# Autodesk Inventor assembly: Top Rail assy
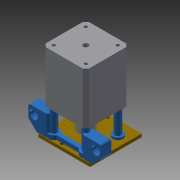
[picture p0: Inventor's stored thumbnail of the model, 180x180]
Saved by Autodesk Inventor 2013 SP2 (Build 170200200, 200)
## iProperties
Created: 2017-01-25
Part Number: Top Rail assy
Document SubType Name: Assembly
Designer: Herman de Vries
Mass: 171.449 g
Surface Area: 753.144 cm^2
Volume: 171.449 cm^3
Density: 1 g/cm^3
Author: Herman de Vries
## Documents named in this file (6)
- C:\Users\hdv\Dropbox\Projects\Inventor\PaintBot_3\Top Rail assy.iam
- C:\Users\hdv\Dropbox\Projects\Inventor\PaintBot_3\Top Rail.ipt
- C:\Users\hdv\Dropbox\Projects\Inventor\PaintBot_3\NEMA42.ipt
- C:\Users\hdv\Dropbox\Projects\Inventor\PaintBot_3\gear belt.ipt
- C:\Users\hdv\Dropbox\Projects\Inventor\PaintBot_3\spacer stepperM.ipt
- C:\Users\hdv\Dropbox\Projects\Inventor\PaintBot_3\spacer stepperM n rail.ipt
## Components (6 placed, 5 different names)
1. Top Rail:1 — Mate:1, Mate:3
2. NEMA42:1 — Insert:1, Mate:1, Mate:3, Insert:5
3. gear belt:1 — Insert:1
4. spacer stepperM:1
5. spacer stepperM:2
6. spacer stepperM n rail:1 — Insert:5
## Relationships (7: Insert 5, Mate 2)
- Insert:1 (5 mm): NEMA42:1 ↔ gear belt:1
- Mate:1 (26 mm): Top Rail:1 ↔ NEMA42:1
- Mate:3: Top Rail:1 ↔ NEMA42:1
- [Insert]: Top Rail:1 ↔ spacer stepperM:1
- [Insert]: Top Rail:1 ↔ spacer stepperM:2
- [Insert]: Top Rail:1 ↔ spacer stepperM n rail:1
- Insert:5: NEMA42:1 ↔ spacer stepperM n rail:1
